# Autodesk Inventor assembly: centergravity
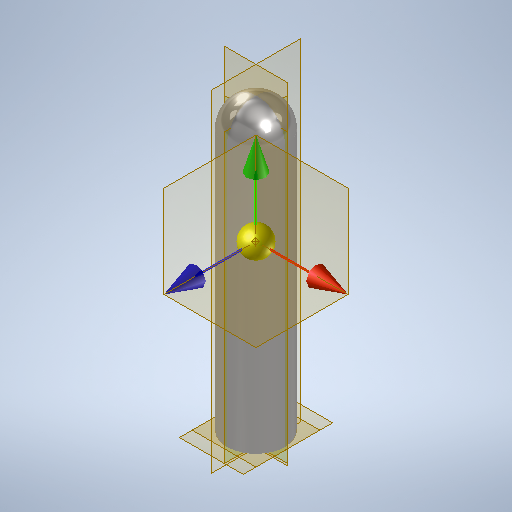
[picture p0: Inventor's stored thumbnail of the model, 512x512]
Saved by Autodesk Inventor 2025.2 (Build 292293000, 293)
## iProperties
Created: 2025-06-19
Part Number: centergravity
Document SubType Name: Assembly
Designer: MSIGAMING
Mass: 128000 g
Surface Area: 11427.5 cm^2
Volume: 16558.8 cm^3
Density: 7.73 g/cm^3
Author: MSIGAMING
## Documents named in this file (3)
- D:\One Drive Manuel\OneDrive\21 Master APE\II Semester\Robotik\3d_robotik\centergravity.iam
- D:\One Drive Manuel\OneDrive\21 Master APE\II Semester\Robotik\3d_robotik\Z1.ipt
- D:\One Drive Manuel\OneDrive\21 Master APE\II Semester\Robotik\3d_robotik\Gelenke.ipt
## Components (2 placed, 2 different names)
1. Z1:1 — Mate:1, Mate:2, Mate:3, Mate:4, Flush:1
2. Gelenke:1 — Mate:1, Mate:2
## Relationships (5: Mate 4, Flush 1)
- Mate:1: Z1:1 ↔ Gelenke:1
- Mate:2: Z1:1 ↔ Gelenke:1
- Mate:3: Z1:1
- Mate:4: Z1:1
- Flush:1: Z1:1
